# Autodesk Inventor assembly: Housing_TOP_ASM
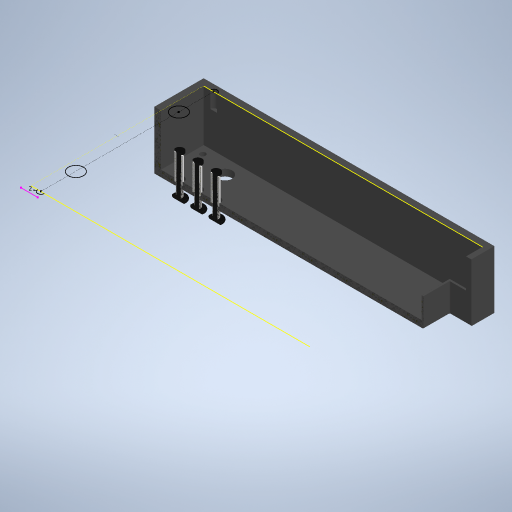
[picture p0: Inventor's stored thumbnail of the model, 512x512]
Saved by Autodesk Inventor 2023.1 (Build 271208000, 208)
## iProperties
Created: 2024-01-10
Part Number: Housing_TOP_ASM
Document SubType Name: Assembly
Designer: JansenL
Author: JansenL
## Documents named in this file (6)
- C:\Users\JansenL\Documents\FHM\Semester_1\ProjektMech\Housing_TOP_ASM.iam
- C:\Users\JansenL\Documents\FHM\Semester_1\ProjektMech\CAD-files\Housing_Top_V2_2.ipt
- C:\Users\JansenL\Documents\FHM\Semester_1\ProjektMech\CAD-files\OLED\938 Mono 128x64 OLED Stemma.iam
- C:\Users\JansenL\Documents\FHM\Semester_1\ProjektMech\CAD-files\TasterAssembled.iam
- C:\Users\JansenL\Documents\FHM\Semester_1\ProjektMech\CAD-files\Fenster_LED.ipt
- C:\Users\JansenL\Documents\FHM\Semester_1\ProjektMech\CAD-files\Fenster_OLED.ipt
## Components (7 placed, 5 different names)
1. Housing_Top_V2_2:1 — Mate:1, Mate:2, Flush:1, Mate:3, Mate:4, Mate:5, Mate:6, Mate:7, Mate:8, Mate:9, Mate:10, Mate:11, Mate:12, Mate:13, Mate:14, Mate:15, Mate:16
2. 938 Mono 128x64 OLED Stemma:1 [sub-assembly] — Mate:3, Mate:4, Mate:5
3. TasterAssembled:1 [sub-assembly] — Mate:6, Mate:10, Flush:2, Flush:3
4. TasterAssembled:2 [sub-assembly] — Mate:7, Mate:11, Flush:2
5. TasterAssembled:3 [sub-assembly] — Mate:8, Mate:9, Flush:3
6. Fenster_LED:1 — Mate:12, Mate:13
7. Fenster_OLED:1 — Mate:14, Mate:15, Mate:16
## Relationships (19: Mate 16, Flush 3)
- Mate:1: Housing_Top_V2_2:1
- Mate:2: Housing_Top_V2_2:1
- Flush:1: Housing_Top_V2_2:1
- Mate:3: Housing_Top_V2_2:1 ↔ 938 Mono 128x64 OLED Stemma:1
- Mate:4 (2 mm): Housing_Top_V2_2:1 ↔ 938 Mono 128x64 OLED Stemma:1
- Mate:5: Housing_Top_V2_2:1 ↔ 938 Mono 128x64 OLED Stemma:1
- Mate:6: Housing_Top_V2_2:1 ↔ TasterAssembled:1
- Mate:7: Housing_Top_V2_2:1 ↔ TasterAssembled:2
- Mate:8: Housing_Top_V2_2:1 ↔ TasterAssembled:3
- Mate:9: Housing_Top_V2_2:1 ↔ TasterAssembled:3
- Mate:10: Housing_Top_V2_2:1 ↔ TasterAssembled:1
- Mate:11: Housing_Top_V2_2:1 ↔ TasterAssembled:2
- Flush:2: TasterAssembled:1 ↔ TasterAssembled:2
- Flush:3: TasterAssembled:1 ↔ TasterAssembled:3
- Mate:12: Housing_Top_V2_2:1 ↔ Fenster_LED:1
- Mate:13: Housing_Top_V2_2:1 ↔ Fenster_LED:1
- Mate:14: Housing_Top_V2_2:1 ↔ Fenster_OLED:1
- Mate:15: Housing_Top_V2_2:1 ↔ Fenster_OLED:1
- Mate:16: Housing_Top_V2_2:1 ↔ Fenster_OLED:1
